# Autodesk Inventor assembly: face
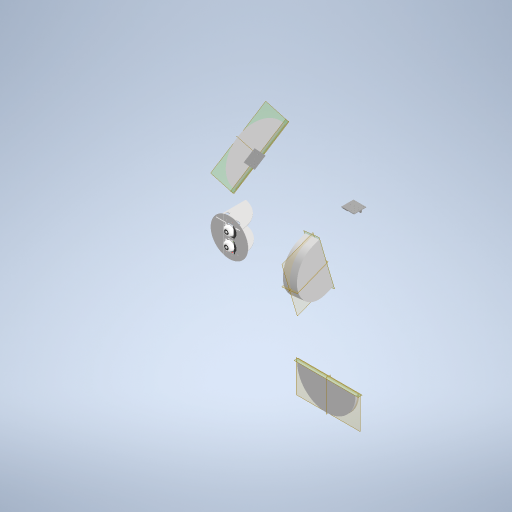
[picture p0: Inventor's stored thumbnail of the model, 512x512]
Saved by Autodesk Inventor 2023.2 (Build 272271030, 271C)
## iProperties
Created: 2024-01-26
Part Number: face
Document SubType Name: Assembly
Designer: I9232
Author: I9232
## Documents named in this file (10)
- D:\!project\fox_n_crow_construction\crow\face\face.iam
- D:\!project\fox_n_crow_construction\crow\face\Сборка глаза вороны.iam
- D:\!project\fox_n_crow_construction\crow\face\Деталь1.ipt
- D:\!project\fox_n_crow_construction\crow\face\Платформа для крыльев лево.ipt
- D:\!project\fox_n_crow_construction\crow\face\Платформа для крыльев право.ipt
- D:\!project\fox_n_crow_construction\crow\face\Сыр.ipt
- D:\!project\fox_n_crow_construction\crow\face\Веер.ipt
- D:\!project\fox_n_crow_construction\crow\face\боковые стороны головы.ipt
- C:\Users\I9232\OneDrive\Рабочий стол\Новая папка\door_hinge.ipt
- D:\!project\fox_n_crow_construction\crow\face\боковые стороны головы_MIR2.ipt
## Components (11 placed, 9 different names)
1. Сборка глаза вороны:1 [sub-assembly] — Заподлицо:1
2. Платформа глаз — Заподлицо:1, Совмещение:1, Совмещение:2, Совмещение:4
3. Платформа для крыльев лево:1
4. Платформа для крыльев право:1 — Жесткий:1
5. Сыр:1
6. Веер:1 — Жесткий:1
7. Веер:2
8. боковые стороны головы:1 — Совмещение:4
9. door_hinge:1 — Совмещение:2
10. door_hinge:2 — Совмещение:1
11. боковые стороны головы_MIR2:1
## Relationships (5: Mate 3, Flush 1, WeldJoint 1)
- Заподлицо:1 [Flush]: Сборка глаза вороны:1 ↔ Платформа глаз
- Жесткий:1 [WeldJoint]: Платформа для крыльев право:1 ↔ Веер:1
- Совмещение:1 [Mate]: Платформа глаз ↔ door_hinge:2
- Совмещение:2 [Mate]: Платформа глаз ↔ door_hinge:1
- Совмещение:4 [Mate]: Платформа глаз ↔ боковые стороны головы:1
